# Autodesk Inventor assembly: Limit Switch (Sensor)
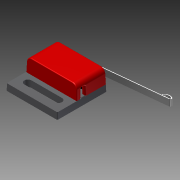
[picture p0: Inventor's stored thumbnail of the model, 180x180]
Saved by Autodesk Inventor 2014 SP1 (Build 180222100, 222)
## iProperties
Created: 2010-04-28
Part Number: Limit Switch (Sensor)
Document SubType Name: Assembly
Designer: Jordan
Mass: 13.608 g
Surface Area: 67.6196 cm^2
Volume: 5.8262 cm^3
Density: 2.33566 g/cm^3
Translation Standard: STEP AP203
FileName: Limit Switch (Sensor).iam
PreProcessor: SolidWorks 2006052
PostProcessor: Build: 239, Release: 2011 RTM - Date: Wed 02/17/2010
Sent Units: inch
Uncertainty: 1e-05
Author: Jordan
## Documents named in this file (4)
- C:\Users\Ryan\Desktop\sw\lib\Super Sonic Sparks VEX CAD Library\Motors & Sensors\Limit Switch (Sensor).iam
- C:\Users\Ryan\Desktop\sw\lib\Super Sonic Sparks VEX CAD Library\Motors & Sensors\Limit Switch (Sensor)-Parts\Top.ipt
- C:\Users\Ryan\Desktop\sw\lib\Super Sonic Sparks VEX CAD Library\Motors & Sensors\Limit Switch (Sensor)-Parts\Microswitch.ipt
- C:\Users\Ryan\Desktop\sw\lib\Super Sonic Sparks VEX CAD Library\Motors & Sensors\Limit Switch (Sensor)-Parts\Bottom.ipt
## Components (3 placed, 3 different names)
1. Top:1
2. Microswitch:1
3. Bottom:1 — Mate:1, Mate:2, Mate:3, Mate:4
## Relationships (4: Mate 4)
- Mate:1 (2.1463 mm): Bottom:1
- Mate:2 (2.1463 mm): Bottom:1
- Mate:3 (15.9611 mm): Bottom:1
- Mate:4 (15.9611 mm): Bottom:1
